# Autodesk Inventor assembly: super_simple
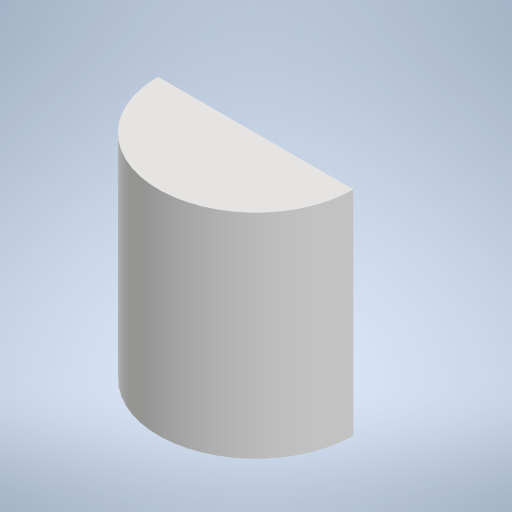
[picture p0: Inventor's stored thumbnail of the model, 512x512]
Saved by Autodesk Inventor 2024 (Build 280153000, 153)
## iProperties
Created: 2023-12-15
Part Number: super_simple
Document SubType Name: Assembly
Designer: dk
Author: dk
## Documents named in this file (3)
- E:\ion_trajectory_integrator\super_simple.iam
- E:\owncloud\BETA_ATLF_H2_Molecular clock (Projectfolder)\05_people\dknapp\007_ion_chamber_assembly\IonTrapKoelemeijVU_Inventor\shield.ipt
- E:\owncloud\BETA_ATLF_H2_Molecular clock (Projectfolder)\05_people\dknapp\007_ion_chamber_assembly\IonTrapKoelemeijVU_Inventor\electrodes.ipt
## Components (2 placed, 2 different names)
1. shield:1 — Flush:1
2. electrodes:1 — Flush:1
## Relationships (1: Flush 1)
- Flush:1 (-85 mm): shield:1 ↔ electrodes:1
